# Autodesk Inventor assembly: Jungheewon
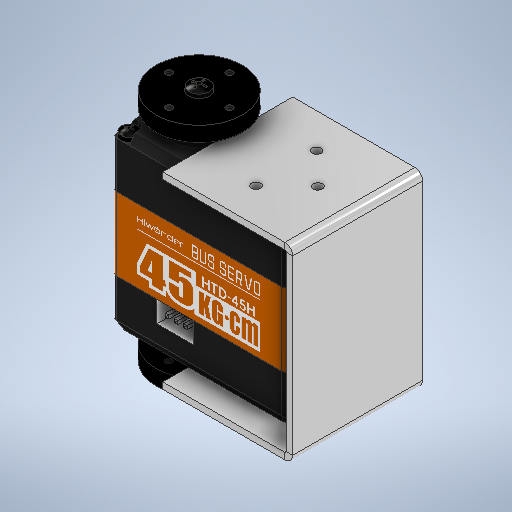
[picture p0: Inventor's stored thumbnail of the model, 512x512]
Saved by Autodesk Inventor 2025.2 (Build 292293000, 293)
## iProperties
Created: 2025-03-25
Part Number: Jungheewon
Document SubType Name: Assembly
Designer: chris
Author: chris
## Documents named in this file (3)
- C:\Users\chris\문서\RH+8 vscode\RHp_hardware_example\Assembly\Jungheewon.iam
- C:\Users\chris\문서\RH+8 vscode\RHp_hardware_example\Part\HTD-45H, Horn\HTD-45H Assembly.iam
- C:\Users\chris\문서\RH+8 vscode\RHp_hardware_example\Part\Frame\chris.ipt
## Components (2 placed, 2 different names)
1. HTD-45H Assembly:1 [sub-assembly] — Flush:1, Flush:2, Flush:3, Flush:4, Mate:1, Mate:2
2. chris:1 — Flush:4, Mate:1, Mate:2
## Relationships (6: Flush 4, Mate 2)
- Flush:1: HTD-45H Assembly:1
- Flush:2: HTD-45H Assembly:1
- Flush:3: HTD-45H Assembly:1
- Flush:4: HTD-45H Assembly:1 ↔ chris:1
- Mate:1: HTD-45H Assembly:1 ↔ chris:1
- Mate:2 (5 mm): HTD-45H Assembly:1 ↔ chris:1
